# Autodesk Inventor assembly: motorAssembly
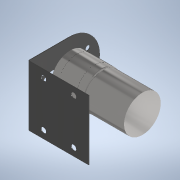
[picture p0: Inventor's stored thumbnail of the model, 180x180]
Saved by Autodesk Inventor 2020 (Build 240168000, 168)
## iProperties
Created: 2022-07-22
Part Number: motorAssembly
Document SubType Name: Assembly
Designer: iPICLab4
Author: iPICLab4
## Documents named in this file (4)
- C:\Users\iPICLab4\Desktop\RG\mech\src\motorAssembly.iam
- C:\Users\iPICLab4\Desktop\RG\mech\src\GearedDCmotor.ipt
- C:\Users\iPICLab4\Desktop\RG\mech\src\motorBracket.ipt
- C:\Users\iPICLab4\Documents\Inventor\Content Center Files\R2020\en-US\AS 1427(01)\AS 1427 - M3 x 5(3).ipt
## Components (4 placed, 3 different names)
1. GearedDCmotor:1 — Mate:1, Mate:6, Mate:7
2. motorBracket:1 — Mate:1, Mate:2, Mate:3, Mate:4, Mate:5
3. AS 1427 - Metric M3 x 5:1 — Mate:2, Mate:5, Mate:6
4. AS 1427 - Metric M3 x 5:2 — Mate:3, Mate:4, Mate:7
## Relationships (7: Mate 7)
- Mate:1: GearedDCmotor:1 ↔ motorBracket:1
- Mate:2: motorBracket:1 ↔ AS 1427 - Metric M3 x 5:1
- Mate:3: motorBracket:1 ↔ AS 1427 - Metric M3 x 5:2
- Mate:4: motorBracket:1 ↔ AS 1427 - Metric M3 x 5:2
- Mate:5: motorBracket:1 ↔ AS 1427 - Metric M3 x 5:1
- Mate:6: GearedDCmotor:1 ↔ AS 1427 - Metric M3 x 5:1
- Mate:7: GearedDCmotor:1 ↔ AS 1427 - Metric M3 x 5:2
